# Autodesk Inventor assembly: H12700ASuppourt
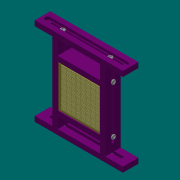
[picture p0: Inventor's stored thumbnail of the model, 180x180]
Saved by Autodesk Inventor 2016 (Build 200138000, 138)
## iProperties
Created: 2015-10-27
Part Number: H12700ASuppourt
Document SubType Name: Assembly
Designer: Sawaiz
Author: Sawaiz
## Documents named in this file (6)
- C:\Users\Sawaiz\OneDrive\projects\modularRICH\H12700A\H12700ASuppourt.iam
- C:\Users\Sawaiz\OneDrive\projects\modularRICH\H12700A\H12700A.iam
- C:\Users\Sawaiz\OneDrive\projects\modularRICH\H12700A\horizontalSupourt.ipt
- C:\Users\Sawaiz\OneDrive\projects\modularRICH\H12700A\verticalSupourt.ipt
- C:\Users\Sawaiz\OneDrive\projects\modularRICH\H12700A\detectorSuppourt.ipt
- C:\Users\Sawaiz\OneDrive\projects\modularRICH\H12700A\4-40x0.325in.ipt
## Components (15 placed, 5 different names)
1. H12700A:1 [sub-assembly] — Flush:1, Flush:4, Flush:5, Mate:4, Mate:5, Flush:7, Mate:6, Mate:7
2. horizontalSupourt:2 — Flush:1, Mate:3, Mate:20, Flush:10, Mate:26, Mate:39
3. verticalSupourt:1 — Flush:5, Mate:5, Mate:20, Mate:23, Mate:27, Mate:32, Mate:35, Mate:37
4. verticalSupourt:2 — Flush:4, Mate:3, Mate:4, Mate:8, Mate:21, Flush:9, Mate:22, Mate:29, Mate:33, Mate:34, Mate:36
5. detectorSuppourt:1 — Flush:6, Flush:7, Mate:6, Flush:8, Mate:30, Mate:31
6. detectorSuppourt:2 — Flush:6, Mate:7, Flush:8, Mate:8, Mate:24, Mate:25
7. horizontalSupourt:3 — Mate:21, Flush:9, Flush:10, Mate:38
8. 4-40x0.325in:1 — Mate:23, Mate:39
9. 4-40x0.325in:2 — Mate:22, Mate:26
10. 4-40x0.325in:3 — Mate:34, Mate:36, Flush:11, Mate:38
11. 4-40x0.325in:4 — Mate:35, Mate:37, Flush:11
12. 4-40x0.325in:5 — Mate:25, Mate:27
13. 4-40x0.325in:6 — Mate:31, Mate:32
14. 4-40x0.325in:7 — Mate:30, Mate:33
15. 4-40x0.325in:8 — Mate:24, Mate:29
## Relationships (34: Mate 25, Flush 9)
- Flush:1: H12700A:1 ↔ horizontalSupourt:2
- Flush:4: H12700A:1 ↔ verticalSupourt:2
- Flush:5: H12700A:1 ↔ verticalSupourt:1
- Mate:3: horizontalSupourt:2 ↔ verticalSupourt:2
- Mate:4: H12700A:1 ↔ verticalSupourt:2
- Mate:5: H12700A:1 ↔ verticalSupourt:1
- Flush:6: detectorSuppourt:1 ↔ detectorSuppourt:2
- Flush:7: H12700A:1 ↔ detectorSuppourt:1
- Mate:6: H12700A:1 ↔ detectorSuppourt:1
- Mate:7: H12700A:1 ↔ detectorSuppourt:2
- Flush:8: detectorSuppourt:1 ↔ detectorSuppourt:2
- Mate:8: verticalSupourt:2 ↔ detectorSuppourt:2
- Mate:20: horizontalSupourt:2 ↔ verticalSupourt:1
- Mate:21: verticalSupourt:2 ↔ horizontalSupourt:3
- Flush:9: verticalSupourt:2 ↔ horizontalSupourt:3
- Flush:10: horizontalSupourt:2 ↔ horizontalSupourt:3
- Mate:22: verticalSupourt:2 ↔ 4-40x0.325in:2
- Mate:23: verticalSupourt:1 ↔ 4-40x0.325in:1
- Mate:24: detectorSuppourt:2 ↔ 4-40x0.325in:8
- Mate:25: detectorSuppourt:2 ↔ 4-40x0.325in:5
- Mate:26: horizontalSupourt:2 ↔ 4-40x0.325in:2
- Mate:27: verticalSupourt:1 ↔ 4-40x0.325in:5
- Mate:29: verticalSupourt:2 ↔ 4-40x0.325in:8
- Mate:30: detectorSuppourt:1 ↔ 4-40x0.325in:7
- Mate:31: detectorSuppourt:1 ↔ 4-40x0.325in:6
- Mate:32: verticalSupourt:1 ↔ 4-40x0.325in:6
- Mate:33: verticalSupourt:2 ↔ 4-40x0.325in:7
- Mate:34: verticalSupourt:2 ↔ 4-40x0.325in:3
- Mate:35: verticalSupourt:1 ↔ 4-40x0.325in:4
- Mate:36: verticalSupourt:2 ↔ 4-40x0.325in:3
- Mate:37: verticalSupourt:1 ↔ 4-40x0.325in:4
- Flush:11: 4-40x0.325in:3 ↔ 4-40x0.325in:4
- Mate:38: horizontalSupourt:3 ↔ 4-40x0.325in:3
- Mate:39: horizontalSupourt:2 ↔ 4-40x0.325in:1
